# Autodesk Inventor assembly: ring_quad_sector4
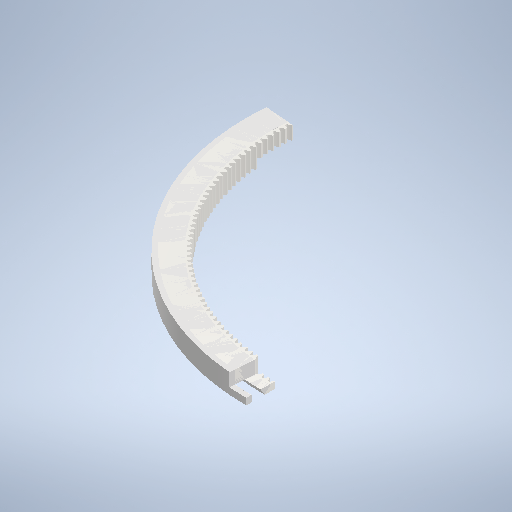
[picture p0: Inventor's stored thumbnail of the model, 512x512]
Saved by Autodesk Inventor 2025 (Build 290162000, 162)
## iProperties
Created: 2025-12-09
Part Number: ring_quad_sector4
Document SubType Name: Assembly
Designer: Admin
Author: Admin
## Documents named in this file (3)
- C:\Users\sum89\OneDrive\Рабочий стол\Ring\Model\ring_quad_sector4.iam
- C:\Users\sum89\OneDrive\Рабочий стол\Ring\Model\assemble_ver4_thick.ipt
- C:\Users\sum89\OneDrive\Рабочий стол\Ring\Model\assemble_ver5_thick\Мастер проектирования\Цилиндрическое зубчатое зацепление1.iam
## Components (2 placed, 2 different names)
1. assemble_ver4_thick:1 — Совмещение:1, Заподлицо:1
2. Цилиндрическое зубчатое зацепление:1 [sub-assembly] — Совмещение:1, Заподлицо:1
## Relationships (2: Mate 1, Flush 1)
- Совмещение:1 [Mate]: assemble_ver4_thick:1 ↔ Цилиндрическое зубчатое зацепление:1
- Заподлицо:1 [Flush]: assemble_ver4_thick:1 ↔ Цилиндрическое зубчатое зацепление:1
